# Autodesk Inventor assembly: Assembly1
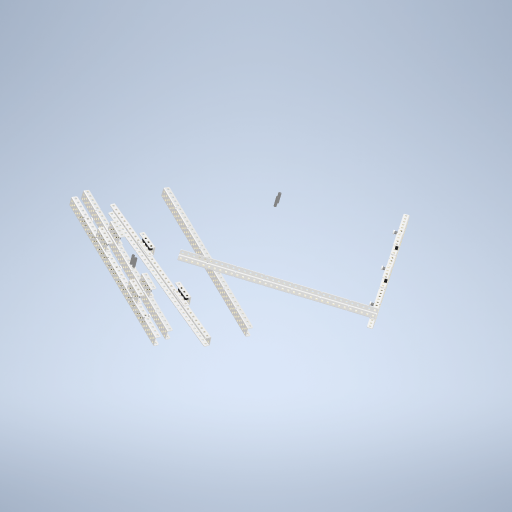
[picture p0: Inventor's stored thumbnail of the model, 512x512]
Saved by Autodesk Inventor 2023.2 (Build 272271000, 271)
## iProperties
Created: 2022-12-13
Part Number: Assembly1
Document SubType Name: Assembly
Designer: 76646426
Author: 76646426
## Documents named in this file (15)
- C:\Users\76646426\Downloads\Assembly1.iam
- C:\Users\Public\Documents\CAD\2021-2022 CAD Library\Structure\C-Channels\Aluminum 1x2x1\Alu C 1x2x1x35.ipt
- C:\Users\Public\Documents\CAD\2021-2022 CAD Library\Motion\Spacers\Spacer Nylon .313 OD\NSpacer .313 OD x .125.ipt
- C:\Users\Public\Documents\CAD\2021-2022 CAD Library\Motion\Spacers\Spacer Nylon .313 OD.ipt
- C:\Users\Public\Documents\CAD\2021-2022 CAD Library\Structure\C-Channels\Aluminum 1x2x1\Alu C 1x2x1x4.ipt
- C:\Users\Public\Documents\CAD\2021-2022 CAD Library\Motion\Bearing Flat.ipt
- C:\Users\76646426\Documents\9691A-Robot-Files\CAD\2021-2022 CAD Library\Structure\Standoff\Standoff 1.00.ipt
- C:\Users\76646426\Documents\9691A-Robot-Files\CAD\2021-2022 CAD Library\Structure\Standoff.ipt
- C:\Users\76646426\Documents\9691A-Robot-Files\CAD\2021-2022 CAD Library\Structure\Standoff\Standoff .50.ipt
- C:\Users\Public\Documents\CAD\2021-2022 CAD Library\Structure\C-Channels\Aluminum 1x2x1\Alu C 1x2x1x35_MIR.ipt
- C:\Users\Public\Documents\CAD\2021-2022 CAD Library\Structure\C-Channels\Aluminum 1x2x1\Alu C 1x2x1x4_MIR.ipt
- C:\Users\Public\Documents\CAD\2021-2022 CAD Library\Motion\Bearing Flat_MIR.ipt
- C:\Users\Public\Documents\CAD\2021-2022 CAD Library\Motion\Bearing Flat_MIR1.ipt
- C:\Users\Public\Documents\CAD\2021-2022 CAD Library\Structure\C-Channels\Aluminum 1x2x1\Alu C 1x2x1x35_MIR1.ipt
- C:\Users\Public\Documents\CAD\2021-2022 CAD Library\Structure\C-Channels\Aluminum 1x2x1\Alu C 1x2x1x4_MIR1.ipt
## Components (67 placed, 12 different names)
1. Alu C 1x2x1x35:1 — Insert:6, Insert:8, Insert:10, Insert:12
2. NSpacer .313 OD x .125:1 — Insert:5, Insert:6
3. NSpacer .313 OD x .125:2 — Insert:7, Insert:8
4. Alu C 1x2x1x4:1 — Insert:3, Insert:4, Insert:5, Insert:7
5. NSpacer .313 OD x .125:3 — Insert:11, Insert:12
6. NSpacer .313 OD x .125:4 — Insert:9, Insert:10
7. Alu C 1x2x1x4:2 — Insert:1, Insert:2, Insert:9, Insert:11
8. Bearing Flat:1 — Insert:1, Insert:2
9. Bearing Flat:2 — Insert:3, Insert:4
10. Bearing Flat:3 — Insert:27, Insert:28
11. Bearing Flat:4 — Insert:21, Insert:22, Insert:23
12. Bearing Flat:5 — Insert:29, Insert:30, Insert:32
13. Bearing Flat:6 — Insert:25, Insert:26
14. Alu C 1x2x1x35:2 — Insert:13, Insert:14, Insert:17, Insert:18, Insert:19, Insert:20, Insert:21, Insert:22, Insert:25, Insert:26, Insert:27, Insert:28, Insert:29, Insert:30
15. NSpacer .313 OD x .125:5
16. NSpacer .313 OD x .125:6
17. Alu C 1x2x1x4:3
18. NSpacer .313 OD x .125:7
19. Alu C 1x2x1x4:4 — Insert:65, Insert:66
20. Bearing Flat:7
21. Standoff 1.00:1
22. Standoff 1.00:2
23. Standoff .50:3 — Insert:15, Insert:16
24. Standoff .50:4 — Insert:23, Insert:24
25. Standoff .50:5 — Insert:31, Insert:32
26. NSpacer .313 OD x .125:8 — Insert:31
27. NSpacer .313 OD x .125:9 — Insert:24
28. NSpacer .313 OD x .125:10 — Insert:16
29. Bearing Flat:8 — Insert:13, Insert:14, Insert:15
30. Bearing Flat:9 — Insert:17, Insert:19
31. Bearing Flat:10 — Insert:18, Insert:20
32. Alu C 1x2x1x35:3 — Insert:81, Insert:82
33. Alu C 1x2x1x35:4
34. Alu C 1x2x1x35_MIR:1 — Insert:33, Insert:34, Insert:37, Insert:38
35. NSpacer .313 OD x .125:11 — Insert:33, Insert:36
36. NSpacer .313 OD x .125:12 — Insert:34, Insert:35
37. Alu C 1x2x1x4_MIR:1 — Insert:35, Insert:36, Insert:43, Insert:44
38. NSpacer .313 OD x .125:13 — Insert:37, Insert:39
39. NSpacer .313 OD x .125:14 — Insert:38, Insert:40
40. Alu C 1x2x1x4_MIR:2 — Insert:39, Insert:40, Insert:41, Insert:42
41. Bearing Flat_MIR:1 — Insert:41, Insert:42
42. Bearing Flat_MIR:2 — Insert:43, Insert:44
43. Bearing Flat_MIR1:1 — Insert:47, Insert:48
44. Bearing Flat_MIR1:2 — Insert:51, Insert:52, Insert:53
45. Bearing Flat_MIR1:3 — Insert:45, Insert:46, Insert:54
46. Bearing Flat_MIR1:4 — Insert:49, Insert:50
47. Alu C 1x2x1x35_MIR1:1 — Insert:45, Insert:46, Insert:47, Insert:48, Insert:49, Insert:50, Insert:51, Insert:52, Insert:59, Insert:60, Insert:61, Insert:62, Insert:63, Insert:64, Insert:79, Insert:80, Insert:81, Insert:82, Insert:83, Insert:84
48. NSpacer .313 OD x .125:15 — Insert:70, Insert:84
49. NSpacer .313 OD x .125:16 — Insert:69, Insert:83
50. Alu C 1x2x1x4_MIR1:1 — Insert:67, Insert:68, Insert:69, Insert:70
51. Bearing Flat_MIR1:5 — Insert:67, Insert:68
52. Standoff 1.00:6
53. Standoff 1.00:7
54. Standoff .50:8 — Insert:57, Insert:58
55. Standoff .50:9 — Insert:53, Insert:56
56. Standoff .50:10 — Insert:54, Insert:55, Mate:58, Mate:59
57. NSpacer .313 OD x .125:18 — Insert:55, Mate:58, Mate:59
58. NSpacer .313 OD x .125:19 — Insert:56
59. NSpacer .313 OD x .125:20 — Insert:57
60. Bearing Flat_MIR1:6 — Insert:58, Insert:59, Insert:60
61. Bearing Flat_MIR1:7 — Insert:61, Insert:62
62. Bearing Flat_MIR1:8 — Insert:63, Insert:64
63. Bearing Flat_MIR1:9 — Insert:65, Insert:66
64. NSpacer .313 OD x .125:21 — Insert:79
65. NSpacer .313 OD x .125:22 — Insert:80
66. Alu C 1x2x1x4_MIR1:2
67. Bearing Flat_MIR1:10
## Relationships (99: Insert 80, Mate 19)
- Insert:1: Alu C 1x2x1x4:2 ↔ Bearing Flat:1
- Insert:2: Alu C 1x2x1x4:2 ↔ Bearing Flat:1
- Insert:3: Alu C 1x2x1x4:1 ↔ Bearing Flat:2
- Insert:4: Alu C 1x2x1x4:1 ↔ Bearing Flat:2
- Insert:5: NSpacer .313 OD x .125:1 ↔ Alu C 1x2x1x4:1
- Insert:6: Alu C 1x2x1x35:1 ↔ NSpacer .313 OD x .125:1
- Insert:7: NSpacer .313 OD x .125:2 ↔ Alu C 1x2x1x4:1
- Insert:8: Alu C 1x2x1x35:1 ↔ NSpacer .313 OD x .125:2
- Insert:9: NSpacer .313 OD x .125:4 ↔ Alu C 1x2x1x4:2
- Insert:10: Alu C 1x2x1x35:1 ↔ NSpacer .313 OD x .125:4
- Insert:11: NSpacer .313 OD x .125:3 ↔ Alu C 1x2x1x4:2
- Insert:12: Alu C 1x2x1x35:1 ↔ NSpacer .313 OD x .125:3
- [Mate]: Alu C 1x2x1x35:2 ↔ NSpacer .313 OD x .125:6
- [Mate]: Alu C 1x2x1x35:2 ↔ NSpacer .313 OD x .125:5
- [Mate]: Alu C 1x2x1x35:2 ↔ NSpacer .313 OD x .125:6
- [Mate]: Alu C 1x2x1x35:2 ↔ NSpacer .313 OD x .125:5
- [Mate]: NSpacer .313 OD x .125:5 ↔ Alu C 1x2x1x4:3
- [Mate]: NSpacer .313 OD x .125:6 ↔ Alu C 1x2x1x4:3
- [Mate]: NSpacer .313 OD x .125:6 ↔ Alu C 1x2x1x4:3
- [Mate]: Alu C 1x2x1x35:2 ↔ NSpacer .313 OD x .125:7
- [Mate]: Alu C 1x2x1x35:2 ↔ NSpacer .313 OD x .125:7
- [Mate]: NSpacer .313 OD x .125:7 ↔ Alu C 1x2x1x4:4
- [Mate]: NSpacer .313 OD x .125:7 ↔ Alu C 1x2x1x4:4
- [Mate]: NSpacer .313 OD x .125:7 ↔ Alu C 1x2x1x4:4
- [Mate]: Alu C 1x2x1x4:3 ↔ Bearing Flat:7
- [Mate]: Alu C 1x2x1x4:3 ↔ Bearing Flat:7
- [Mate]: Alu C 1x2x1x4:3 ↔ Bearing Flat:7
- [Mate]: Standoff .50:5 ↔ NSpacer .313 OD x .125:8
- [Mate]: Standoff .50:5 ↔ NSpacer .313 OD x .125:8
- Insert:13: Alu C 1x2x1x35:2 ↔ Bearing Flat:8
- Insert:14: Alu C 1x2x1x35:2 ↔ Bearing Flat:8
- Insert:15: Standoff .50:3 ↔ Bearing Flat:8
- Insert:16: Standoff .50:3 ↔ NSpacer .313 OD x .125:10
- Insert:17: Alu C 1x2x1x35:2 ↔ Bearing Flat:9
- Insert:18: Alu C 1x2x1x35:2 ↔ Bearing Flat:10
- Insert:19: Alu C 1x2x1x35:2 ↔ Bearing Flat:9
- Insert:20: Alu C 1x2x1x35:2 ↔ Bearing Flat:10
- Insert:21: Bearing Flat:4 ↔ Alu C 1x2x1x35:2
- Insert:22: Bearing Flat:4 ↔ Alu C 1x2x1x35:2
- Insert:23: Bearing Flat:4 ↔ Standoff .50:4
- Insert:24: Standoff .50:4 ↔ NSpacer .313 OD x .125:9
- Insert:25: Bearing Flat:6 ↔ Alu C 1x2x1x35:2
- Insert:26: Bearing Flat:6 ↔ Alu C 1x2x1x35:2
- Insert:27: Bearing Flat:3 ↔ Alu C 1x2x1x35:2
- Insert:28: Bearing Flat:3 ↔ Alu C 1x2x1x35:2
- Insert:29: Bearing Flat:5 ↔ Alu C 1x2x1x35:2
- Insert:30: Bearing Flat:5 ↔ Alu C 1x2x1x35:2
- Insert:31: Standoff .50:5 ↔ NSpacer .313 OD x .125:8
- Insert:32: Bearing Flat:5 ↔ Standoff .50:5
- Insert:33: Alu C 1x2x1x35_MIR:1 ↔ NSpacer .313 OD x .125:11
- Insert:34: Alu C 1x2x1x35_MIR:1 ↔ NSpacer .313 OD x .125:12
- Insert:35: NSpacer .313 OD x .125:12 ↔ Alu C 1x2x1x4_MIR:1
- Insert:36: NSpacer .313 OD x .125:11 ↔ Alu C 1x2x1x4_MIR:1
- Insert:37: Alu C 1x2x1x35_MIR:1 ↔ NSpacer .313 OD x .125:13
- Insert:38: Alu C 1x2x1x35_MIR:1 ↔ NSpacer .313 OD x .125:14
- Insert:39: NSpacer .313 OD x .125:13 ↔ Alu C 1x2x1x4_MIR:2
- Insert:40: NSpacer .313 OD x .125:14 ↔ Alu C 1x2x1x4_MIR:2
- Insert:41: Alu C 1x2x1x4_MIR:2 ↔ Bearing Flat_MIR:1
- Insert:42: Alu C 1x2x1x4_MIR:2 ↔ Bearing Flat_MIR:1
- Insert:43: Alu C 1x2x1x4_MIR:1 ↔ Bearing Flat_MIR:2
- Insert:44: Alu C 1x2x1x4_MIR:1 ↔ Bearing Flat_MIR:2
- Insert:45: Bearing Flat_MIR1:3 ↔ Alu C 1x2x1x35_MIR1:1
- Insert:46: Bearing Flat_MIR1:3 ↔ Alu C 1x2x1x35_MIR1:1
- Insert:47: Bearing Flat_MIR1:1 ↔ Alu C 1x2x1x35_MIR1:1
- Insert:48: Bearing Flat_MIR1:1 ↔ Alu C 1x2x1x35_MIR1:1
- Insert:49: Bearing Flat_MIR1:4 ↔ Alu C 1x2x1x35_MIR1:1
- Insert:50: Bearing Flat_MIR1:4 ↔ Alu C 1x2x1x35_MIR1:1
- Insert:51: Bearing Flat_MIR1:2 ↔ Alu C 1x2x1x35_MIR1:1
- Insert:52: Bearing Flat_MIR1:2 ↔ Alu C 1x2x1x35_MIR1:1
- Insert:53: Bearing Flat_MIR1:2 ↔ Standoff .50:9
- Insert:54: Bearing Flat_MIR1:3 ↔ Standoff .50:10
- Insert:55: Standoff .50:10 ↔ NSpacer .313 OD x .125:18
- Mate:58: Standoff .50:10 ↔ NSpacer .313 OD x .125:18
- Mate:59: Standoff .50:10 ↔ NSpacer .313 OD x .125:18
- Insert:56: Standoff .50:9 ↔ NSpacer .313 OD x .125:19
- Insert:57: Standoff .50:8 ↔ NSpacer .313 OD x .125:20
- Insert:58: Standoff .50:8 ↔ Bearing Flat_MIR1:6
- Insert:59: Alu C 1x2x1x35_MIR1:1 ↔ Bearing Flat_MIR1:6
- Insert:60: Alu C 1x2x1x35_MIR1:1 ↔ Bearing Flat_MIR1:6
- Insert:61: Alu C 1x2x1x35_MIR1:1 ↔ Bearing Flat_MIR1:7
- Insert:62: Alu C 1x2x1x35_MIR1:1 ↔ Bearing Flat_MIR1:7
- Insert:63: Alu C 1x2x1x35_MIR1:1 ↔ Bearing Flat_MIR1:8
- Insert:64: Alu C 1x2x1x35_MIR1:1 ↔ Bearing Flat_MIR1:8
- Insert:65: Alu C 1x2x1x4:4 ↔ Bearing Flat_MIR1:9
- Insert:66: Alu C 1x2x1x4:4 ↔ Bearing Flat_MIR1:9
- Insert:67: Alu C 1x2x1x4_MIR1:1 ↔ Bearing Flat_MIR1:5
- Insert:68: Alu C 1x2x1x4_MIR1:1 ↔ Bearing Flat_MIR1:5
- Insert:69: NSpacer .313 OD x .125:16 ↔ Alu C 1x2x1x4_MIR1:1
- Insert:70: NSpacer .313 OD x .125:15 ↔ Alu C 1x2x1x4_MIR1:1
- [Insert]: Alu C 1x2x1x4_MIR1:2 ↔ Bearing Flat_MIR1:10
- [Insert]: Alu C 1x2x1x4_MIR1:2 ↔ Bearing Flat_MIR1:10
- [Insert]: NSpacer .313 OD x .125:22 ↔ Alu C 1x2x1x4_MIR1:2
- [Insert]: NSpacer .313 OD x .125:21 ↔ Alu C 1x2x1x4_MIR1:2
- Insert:79: Alu C 1x2x1x35_MIR1:1 ↔ NSpacer .313 OD x .125:21
- Insert:80: Alu C 1x2x1x35_MIR1:1 ↔ NSpacer .313 OD x .125:22
- Insert:81: Alu C 1x2x1x35:3 ↔ Alu C 1x2x1x35_MIR1:1
- Insert:82: Alu C 1x2x1x35:3 ↔ Alu C 1x2x1x35_MIR1:1
- Insert:83: Alu C 1x2x1x35_MIR1:1 ↔ NSpacer .313 OD x .125:16
- Insert:84: Alu C 1x2x1x35_MIR1:1 ↔ NSpacer .313 OD x .125:15
## Named parameters: d206_d202 = 0 mm, d207_d203 = 0 mm, d208_d204 = 0 mm, d209_d205 = 0 mm
